# Autodesk Inventor assembly: VoiceCoil_Assembly
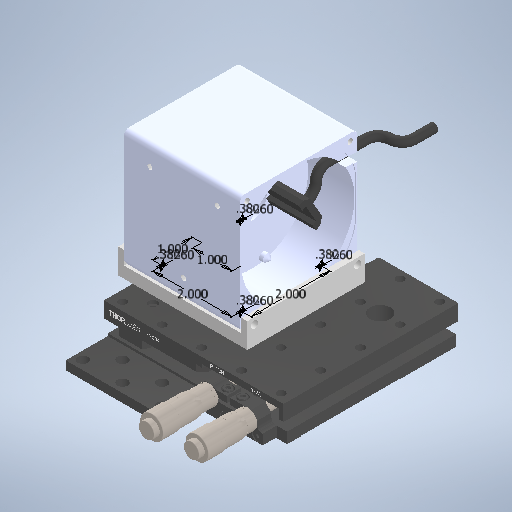
[picture p0: Inventor's stored thumbnail of the model, 512x512]
Saved by Autodesk Inventor 2025.2 (Build 292293000, 293)
## iProperties
Created: 2024-11-27
Part Number: VoiceCoil_Assembly
Document SubType Name: Assembly
Designer: monolithic
Author: monolithic
## Documents named in this file (4)
- C:\Users\monolithic\Documents\GitHub\CAD\Monolith\John\Altair_PowellBaseplate_SPIM_ASLM_CTASLM\Assembly\SubAssemblies\VoiceCoil_Assembly.iam
- C:\Users\monolithic\Documents\GitHub\CAD\Monolith\John\Altair_PowellBaseplate_SPIM_ASLM_CTASLM\Assembly\SubAssemblies\PY004-Step.ipt
- C:\Users\monolithic\Documents\GitHub\CAD\Monolith\John\Altair_PowellBaseplate_SPIM_ASLM_CTASLM\Assembly\SubAssemblies\Voicecoil_to_PY004_Coupler.ipt
- C:\Users\monolithic\Documents\GitHub\CAD\Monolith\John\Altair_PowellBaseplate_SPIM_ASLM_CTASLM\Assembly\SubAssemblies\LFA-2010.ipt
## Components (3 placed, 3 different names)
1. PY004-Step:1 — Mate:1, Angle:1, Mate:6
2. Voicecoil_to_PY004_Coupler:1 — Mate:1, Angle:1, Mate:3, Mate:4, Mate:5, Mate:6
3. LFA-2010:1 — Mate:3, Mate:4, Mate:5
## Relationships (6: Mate 5, Angle 1)
- Mate:1: PY004-Step:1 ↔ Voicecoil_to_PY004_Coupler:1
- Angle:1 (0 deg): PY004-Step:1 ↔ Voicecoil_to_PY004_Coupler:1
- Mate:3: Voicecoil_to_PY004_Coupler:1 ↔ LFA-2010:1
- Mate:4: Voicecoil_to_PY004_Coupler:1 ↔ LFA-2010:1
- Mate:5: Voicecoil_to_PY004_Coupler:1 ↔ LFA-2010:1
- Mate:6: PY004-Step:1 ↔ Voicecoil_to_PY004_Coupler:1
